# Autodesk Inventor assembly: manifold assembly
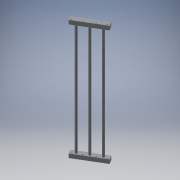
[picture p0: Inventor's stored thumbnail of the model, 180x180]
Saved by Autodesk Inventor 2018 (Build 220112000, 112)
## iProperties
Created: 2018-06-18
Part Number: manifold assembly
Document SubType Name: Assembly
Designer: John Viljoen
Author: John Viljoen
## Documents named in this file (3)
- C:\Users\John Viljoen\Documents\Inventor\computer project\manifold assembly.iam
- C:\Users\John Viljoen\Documents\Inventor\computer project\manifold mirror.ipt
- C:\Users\John Viljoen\Documents\Inventor\computer project\coverplate pipe.ipt
## Components (5 placed, 2 different names)
1. manifold mirror:1 — Mate:1, Mate:2, Mate:6, Mate:7, Mate:8, Mate:9
2. coverplate pipe:1 — Mate:5, Mate:6, Mate:7
3. coverplate pipe:2 — Mate:1, Mate:2, Mate:3, Mate:10
4. coverplate pipe:3 — Mate:8, Mate:9
5. manifold mirror:2 — Mate:3, Mate:5, Mate:10
## Relationships (9: Mate 9)
- Mate:1: manifold mirror:1 ↔ coverplate pipe:2
- Mate:2 (-0.5 mm): manifold mirror:1 ↔ coverplate pipe:2
- Mate:3: coverplate pipe:2 ↔ manifold mirror:2
- Mate:5: coverplate pipe:1 ↔ manifold mirror:2
- Mate:6 (-0.5 mm): manifold mirror:1 ↔ coverplate pipe:1
- Mate:7: manifold mirror:1 ↔ coverplate pipe:1
- Mate:8: manifold mirror:1 ↔ coverplate pipe:3
- Mate:9 (-0.5 mm): manifold mirror:1 ↔ coverplate pipe:3
- Mate:10 (-0.5 mm): coverplate pipe:2 ↔ manifold mirror:2
